# Autodesk Inventor assembly: Arm 2 Assembly
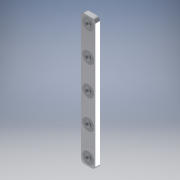
[picture p0: Inventor's stored thumbnail of the model, 180x180]
Saved by Autodesk Inventor 2016 (Build 200138000, 138)
## iProperties
Created: 2015-07-08
Part Number: Arm 2 Assembly
Document SubType Name: Assembly
Designer: Dennis
Author: Dennis
## Documents named in this file (3)
- C:\Users\Matthew Cheung\Dropbox\Work\National Instruments\Shared Folder\NI Ball Bearing Slider Crank\CAD\Assemblies\Arm 2 Assembly.iam
- C:\Users\Matthew Cheung\Dropbox\Work\National Instruments\Shared Folder\NI Ball Bearing Slider Crank\CAD\Arm 2.ipt
- C:\Users\Matthew Cheung\Dropbox\Work\National Instruments\Shared Folder\NI Ball Bearing Slider Crank\CAD\Bearing - 6384K342.ipt
## Components (6 placed, 2 different names)
1. Arm 2:1 — Mate:1, Mate:3, Mate:4, Mate:5, Mate:6, Mate:7, Mate:8, Mate:9, Mate:10, Mate:11
2. Bearing - 6384K342:1 — Mate:1, Mate:3
3. Bearing - 6384K342:2 — Mate:4, Mate:5
4. Bearing - 6384K342:3 — Mate:6, Mate:7
5. Bearing - 6384K342:4 — Mate:10, Mate:11
6. Bearing - 6384K342:5 — Mate:8, Mate:9
## Relationships (10: Mate 10)
- Mate:1: Arm 2:1 ↔ Bearing - 6384K342:1
- Mate:3: Arm 2:1 ↔ Bearing - 6384K342:1
- Mate:4: Arm 2:1 ↔ Bearing - 6384K342:2
- Mate:5: Arm 2:1 ↔ Bearing - 6384K342:2
- Mate:6: Arm 2:1 ↔ Bearing - 6384K342:3
- Mate:7: Arm 2:1 ↔ Bearing - 6384K342:3
- Mate:8: Arm 2:1 ↔ Bearing - 6384K342:5
- Mate:9: Arm 2:1 ↔ Bearing - 6384K342:5
- Mate:10: Arm 2:1 ↔ Bearing - 6384K342:4
- Mate:11: Arm 2:1 ↔ Bearing - 6384K342:4
